# Autodesk Inventor assembly: (FINAL)rollerAssembly
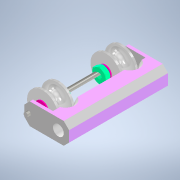
[picture p0: Inventor's stored thumbnail of the model, 180x180]
Saved by Autodesk Inventor 2022 (Build 260153000, 153)
## iProperties
Created: 2022-11-15
Part Number: (FINAL)rollerAssembly
Document SubType Name: Assembly
Designer: matia
Author: matia
## Documents named in this file (7)
- C:\Users\natha\Documents\GitHub\RelativityProjUMD\(V2) FULL ASSEMBLY\(FINAL)rollerAssembly.iam
- C:\Users\natha\Documents\GitHub\RelativityProjUMD\(V2) FULL ASSEMBLY\rollerbase(v2).ipt
- C:\Users\natha\Documents\GitHub\RelativityProjUMD\(V2) FULL ASSEMBLY\wheel.ipt
- C:\Users\natha\Documents\GitHub\RelativityProjUMD\(V2) FULL ASSEMBLY\wheelbushing.ipt
- C:\Users\natha\Documents\GitHub\RelativityProjUMD\(V2) FULL ASSEMBLY\rollerwasher.ipt
- C:\Users\natha\Documents\GitHub\RelativityProjUMD\(V2) FULL ASSEMBLY\90480A006_Low-Strength Steel Hex Nut (.125).ipt
- C:\Users\natha\Documents\GitHub\RelativityProjUMD\(V2) FULL ASSEMBLY\new 18-8 axle.ipt
## Components (12 placed, 6 different names)
1. rollerbase(v2):1 — Insert:1
2. wheel:1 — Mate:11, Mate:12
3. wheel:2 — Mate:13, Mate:14
4. wheelbushing:1 — Mate:11, Mate:12
5. wheelbushing:2 — Mate:13, Mate:14
6. rollerwasher:1
7. rollerwasher:2
8. rollerwasher:3
9. rollerwasher:4
10. 90480A006_Low-Strength Steel Hex Nut (.125):1
11. 90480A006_Low-Strength Steel Hex Nut (.125):2
12. new 18-8 axle:1 — Insert:1
## Relationships (5: Mate 4, Insert 1)
- Mate:11: wheel:1 ↔ wheelbushing:1
- Mate:12: wheel:1 ↔ wheelbushing:1
- Mate:13: wheel:2 ↔ wheelbushing:2
- Mate:14: wheel:2 ↔ wheelbushing:2
- Insert:1 (-3.175 mm): rollerbase(v2):1 ↔ new 18-8 axle:1
